# Autodesk Inventor assembly: Assembly1
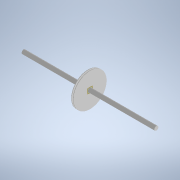
[picture p0: Inventor's stored thumbnail of the model, 180x180]
Saved by Autodesk Inventor 2021 (Build 250183000, 183)
## iProperties
Created: 2021-05-31
Part Number: Assembly1
Document SubType Name: Assembly
Designer: techv
Author: techv
## Documents named in this file (3)
- D:\Projects\P_E Transmision\Design\Assembly1.iam
- D:\Projects\P_E Transmision\Design\Base Plate.ipt
- D:\Projects\P_E Transmision\Design\Shaft.ipt
## Components (2 placed, 2 different names)
1. Base Plate:1 — Mate:1
2. Shaft:1 — Flush:1
## Relationships (2: Flush 1, Mate 1)
- Flush:1 (-500 mm): Shaft:1
- Mate:1: Base Plate:1
